# Autodesk Inventor assembly: cutter_assembly
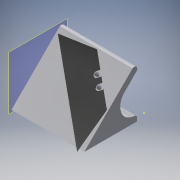
[picture p0: Inventor's stored thumbnail of the model, 180x180]
Saved by Autodesk Inventor 2019 (Build 230136000, 136)
## iProperties
Created: 2019-03-02
Part Number: cutter_assembly
Document SubType Name: Assembly
Designer: assman
Author: assman
## Documents named in this file (3)
- D:\Inventor\Projects\Cutter\cutter_assembly.iam
- D:\Inventor\Projects\Cutter\cutter.ipt
- D:\Inventor\Projects\Cutter\blade.ipt
## Components (2 placed, 2 different names)
1. cutter:1 — Rotational:2
2. blade:1 — Rotational:2
## Relationships (1: RevoluteJoint 1)
- Rotational:2 [RevoluteJoint]: cutter:1 ↔ blade:1
